# Autodesk Inventor assembly: robot
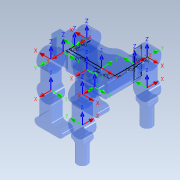
[picture p0: Inventor's stored thumbnail of the model, 180x180]
Saved by Autodesk Inventor 2020 (Build 240168000, 168)
## iProperties
Created: 2021-01-29
Part Number: robot
Document SubType Name: Assembly
Designer: DELL
Author: DELL
## Documents named in this file (6)
- F:\SoftRobot2.0\FlexipodFast\mesh\v9.0\robot.iam
- F:\SoftRobot2.0\FlexipodFast\mesh\v9.0\hip.ipt
- F:\SoftRobot2.0\FlexipodFast\mesh\v9.0\thigh.ipt
- F:\SoftRobot2.0\FlexipodFast\mesh\v9.0\shank_2.ipt
- F:\SoftRobot2.0\FlexipodFast\mesh\v9.0\shank_front.ipt
- F:\SoftRobot2.0\FlexipodFast\mesh\v9.0\body.ipt
## Components (13 placed, 5 different names)
1. hip:1 — Flush:45, Mate:54, Mate:60, Mate:61, Angle:23
2. hip:2 — Angle:22, Mate:52, Mate:53, Mate:58, Mate:59, Angle:26
3. thigh:1 — Mate:44, Flush:43, Mate:52, Mate:53, Angle:27
4. thigh:2 — Mate:43, Flush:42, Flush:45, Mate:54, Angle:24
5. thigh:3 — Mate:42, Flush:41, Mate:55, Mate:56, Angle:33
6. thigh:4 — Mate:41, Flush:40, Mate:57, Flush:46, Angle:30
7. shank_2:3 — Mate:41, Flush:40, Angle:31
8. shank_2:4 — Mate:42, Flush:41, Angle:34
9. shank_front:1 — Mate:43, Flush:42, Angle:25
10. shank_front:2 — Mate:44, Flush:43, Angle:22, Angle:28
11. hip:3 — Mate:55, Mate:56, Mate:65, Mate:66, Angle:32
12. hip:4 — Mate:57, Flush:46, Mate:62, Mate:63, Angle:29, Mate:64, Mate:66
13. body:1 — Flush:47, Flush:48, Flush:49, Mate:58, Mate:59, Mate:60, Mate:61, Angle:23, Angle:24, Angle:25, Angle:26, Angle:27, Angle:28, Mate:62, Mate:63, Angle:29, Angle:30, Angle:31, Mate:64, Mate:65, Angle:32, Angle:33, Angle:34
## Relationships (41: Mate 19, Angle 13, Flush 9)
- Mate:41: thigh:4 ↔ shank_2:3
- Flush:40: thigh:4 ↔ shank_2:3
- Mate:42: thigh:3 ↔ shank_2:4
- Flush:41: thigh:3 ↔ shank_2:4
- Mate:43: thigh:2 ↔ shank_front:1
- Mate:44: thigh:1 ↔ shank_front:2
- Flush:42: thigh:2 ↔ shank_front:1
- Flush:43: thigh:1 ↔ shank_front:2
- Angle:22 (180 deg): hip:2 ↔ shank_front:2
- Mate:52: hip:2 ↔ thigh:1
- Mate:53: hip:2 ↔ thigh:1
- Flush:45: hip:1 ↔ thigh:2
- Mate:54: hip:1 ↔ thigh:2
- Mate:55: thigh:3 ↔ hip:3
- Mate:56: thigh:3 ↔ hip:3
- Mate:57: thigh:4 ↔ hip:4
- Flush:46: thigh:4 ↔ hip:4
- Flush:47: body:1
- Flush:48: body:1
- Flush:49: body:1
- Mate:58: hip:2 ↔ body:1
- Mate:59: hip:2 ↔ body:1
- Mate:60: hip:1 ↔ body:1
- Mate:61: hip:1 ↔ body:1
- Angle:23 (0 deg): hip:1 ↔ body:1
- Angle:24 (0 deg): thigh:2 ↔ body:1
- Angle:25 (0 deg): shank_front:1 ↔ body:1
- Angle:26 (0 deg): hip:2 ↔ body:1
- Angle:27 (0 deg): thigh:1 ↔ body:1
- Angle:28 (0 deg): shank_front:2 ↔ body:1
- Mate:62 (-5 mm): hip:4 ↔ body:1
- Mate:63: hip:4 ↔ body:1
- Angle:29 (0 deg): hip:4 ↔ body:1
- Angle:30 (0 deg): thigh:4 ↔ body:1
- Angle:31 (0 deg): shank_2:3 ↔ body:1
- Mate:64 (-71 mm): hip:4 ↔ body:1
- Mate:65 (-5 mm): hip:3 ↔ body:1
- Mate:66: hip:3 ↔ hip:4
- Angle:32 (0 deg): hip:3 ↔ body:1
- Angle:33 (0 deg): thigh:3 ↔ body:1
- Angle:34 (0 deg): shank_2:4 ↔ body:1
